# Autodesk Inventor assembly: Assembly1
(part 6 of 8)
- Mate:990: FRAME:1 ↔ disk holder:41
- Mate:991: FRAME:1 ↔ disk holder:41
- Mate:992: FRAME:1 ↔ disk holder:39
- Mate:993: FRAME:1 ↔ disk holder:39
- Mate:994: FRAME:1 ↔ disk holder:40
- Mate:995: FRAME:1 ↔ disk holder:40
- Mate:996: FRAME:1 ↔ disk holder:15
- Mate:997: FRAME:1 ↔ disk holder:13
- Mate:998: FRAME:1 ↔ disk holder:36
- Mate:999: FRAME:1 ↔ disk holder:36
- Mate:1000: FRAME:1 ↔ disk holder:37
- Mate:1001: FRAME:1 ↔ disk holder:37
- Mate:1002: FRAME:1 ↔ disk holder:35
- Mate:1003: FRAME:1 ↔ disk holder:35
- Mate:1004: FRAME:1 ↔ disk holder:27
- Mate:1005: FRAME:1 ↔ disk holder:27
- Mate:1006: FRAME:1 ↔ disk holder:30
- Mate:1007: FRAME:1 ↔ disk holder:30
- Mate:1008: FRAME:1 ↔ disk holder:26
- Mate:1009: FRAME:1 ↔ disk holder:26
- Mate:1010: FRAME:1 ↔ disk holder:48
- Mate:1011: FRAME:1 ↔ disk holder:47
- [RevoluteJoint]: disk holder:179 ↔ coin:179
- [Angle] (-25 deg): disk holder:179 ↔ coin:179
- [Mate]: disk holder:179 ↔ Coil:357
- [Mate]: disk holder:179 ↔ Coil:357
- [Angle] (270 deg): disk holder:179 ↔ Coil:357
- [Mate]: disk holder:179 ↔ Coil:358
- [Angle] (270 deg): disk holder:179 ↔ Coil:358
- [Mate]: disk holder:179 ↔ Coil:358
- Flush:274: FRAME:1 ↔ disk holder:179
- Mate:1016: FRAME:1 ↔ disk holder:179
- Mate:1017: FRAME:1 ↔ disk holder:179
- [RevoluteJoint]: disk holder:180 ↔ coin:180
- [Angle] (-25 deg): disk holder:180 ↔ coin:180
- [Mate]: disk holder:180 ↔ Coil:359
- [Mate]: disk holder:180 ↔ Coil:359
- [Angle] (270 deg): disk holder:180 ↔ Coil:359
- [Mate]: disk holder:180 ↔ Coil:360
- [Angle] (270 deg): disk holder:180 ↔ Coil:360
- [Mate]: disk holder:180 ↔ Coil:360
- [RevoluteJoint]: disk holder:181 ↔ coin:181
- [Angle] (-25 deg): disk holder:181 ↔ coin:181
- [Mate]: disk holder:181 ↔ Coil:361
- [Mate]: disk holder:181 ↔ Coil:361
- [Angle] (270 deg): disk holder:181 ↔ Coil:361
- [Mate]: disk holder:181 ↔ Coil:362
- [Angle] (270 deg): disk holder:181 ↔ Coil:362
- [Mate]: disk holder:181 ↔ Coil:362
- [RevoluteJoint]: disk holder:182 ↔ coin:182
- [Angle] (-25 deg): disk holder:182 ↔ coin:182
- [Mate]: disk holder:182 ↔ Coil:363
- [Mate]: disk holder:182 ↔ Coil:363
- [Angle] (270 deg): disk holder:182 ↔ Coil:363
- [Mate]: disk holder:182 ↔ Coil:364
- [Angle] (270 deg): disk holder:182 ↔ Coil:364
- [Mate]: disk holder:182 ↔ Coil:364
- [RevoluteJoint]: disk holder:183 ↔ coin:183
- [Angle] (-25 deg): disk holder:183 ↔ coin:183
- [Mate]: disk holder:183 ↔ Coil:365
- [Mate]: disk holder:183 ↔ Coil:365
- [Angle] (270 deg): disk holder:183 ↔ Coil:365
- [Mate]: disk holder:183 ↔ Coil:366
- [Angle] (270 deg): disk holder:183 ↔ Coil:366
- [Mate]: disk holder:183 ↔ Coil:366
- Flush:275: disk holder:182 ↔ disk holder:183
- Flush:276: disk holder:181 ↔ disk holder:182
- Flush:277: disk holder:180 ↔ disk holder:183
- Flush:278: disk holder:182 ↔ disk holder:183
- Flush:279: disk holder:181 ↔ disk holder:182
- Flush:280: disk holder:180 ↔ disk holder:181
- Mate:1034: FRAME:1 ↔ disk holder:180
- Mate:1035: FRAME:1 ↔ disk holder:181
- Mate:1036: FRAME:1 ↔ disk holder:182
- Mate:1037: FRAME:1 ↔ disk holder:183
- Mate:1038: FRAME:1 ↔ disk holder:180